# Autodesk Inventor assembly: Mouse
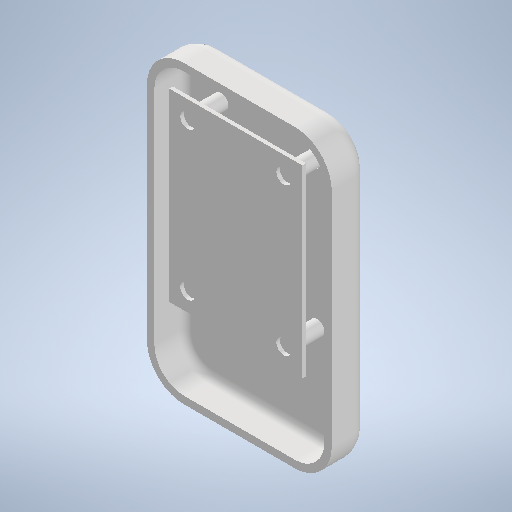
[picture p0: Inventor's stored thumbnail of the model, 512x512]
Saved by Autodesk Inventor 2025 (Build 290162010, 162A)
## iProperties
Created: 2025-10-21
Part Number: Mouse
Document SubType Name: Assembly
Designer: 202321250026
Author: 202321250026
## Documents named in this file (3)
- D:\Users\202321250026\Documents\Github\eng-comp\desenho-assistido\Inventor\Aula_02\Mouse.iam
- D:\Users\202321250026\Documents\Github\eng-comp\desenho-assistido\Inventor\Aula_02\Carcaca-Baixa.ipt
- D:\Users\202321250026\Documents\Github\eng-comp\desenho-assistido\Inventor\Aula_02\Placa-Circuito.ipt
## Components (2 placed, 2 different names)
1. Carcaca-Baixa:1 — Alinhado:1
2. Placa-Circuito:1 — Alinhado:1
## Relationships (1: Flush 1)
- Alinhado:1 [Flush]: Carcaca-Baixa:1 ↔ Placa-Circuito:1
